# Autodesk Inventor assembly: perception module
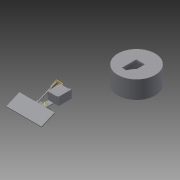
[picture p0: Inventor's stored thumbnail of the model, 180x180]
Saved by Autodesk Inventor 2015 (Build 190159000, 159)
## iProperties
Created: 2014-10-20
Part Number: perception module
Document SubType Name: Assembly
Designer: ericd_000
Author: ericd_000
## Documents named in this file (5)
- C:\Users\ericd_000\Dropbox\GitHub\initial_cad\eric_cad\perception module.iam
- C:\Users\ericd_000\Dropbox\GitHub\initial_cad\eric_cad\herkulex assembled.iam
- C:\Users\ericd_000\Dropbox\GitHub\initial_cad\eric_cad\per_base.ipt
- C:\Users\ericd_000\Dropbox\GitHub\initial_cad\eric_cad\first_perc_link.ipt
- C:\Users\ericd_000\Dropbox\GitHub\initial_cad\eric_cad\second_perc_link.ipt
## Components (5 placed, 4 different names)
1. herkulex assembled:1 [sub-assembly] — Mate:2, Rotational:1, Mate:3, Mate:4
2. herkulex assembled:2 [sub-assembly] — Mate:1
3. per_base:1
4. first_perc_link:1 — Mate:1, Mate:2, Rotational:1
5. second_perc_link:1 — Mate:3, Mate:4
## Relationships (5: Mate 4, RevoluteJoint 1)
- Mate:1: herkulex assembled:2 ↔ first_perc_link:1
- Mate:2: herkulex assembled:1 ↔ first_perc_link:1
- Rotational:1 [RevoluteJoint]: herkulex assembled:1 ↔ first_perc_link:1
- Mate:3: herkulex assembled:1 ↔ second_perc_link:1
- Mate:4: herkulex assembled:1 ↔ second_perc_link:1
